# Autodesk Inventor assembly: Knee
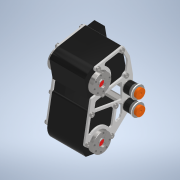
[picture p0: Inventor's stored thumbnail of the model, 180x180]
Saved by Autodesk Inventor 2020 (Build 240168000, 168)
## iProperties
Created: 2022-06-14
Part Number: Knee
Document SubType Name: Assembly
Designer: Masato Kubotera
Author: Masato Kubotera
## Documents named in this file (12)
- C:\Users\MasatoKubotera\Documents\Inventor\SUSTAINA-OP\LowerBody\Knee\Knee.iam
- C:\Users\MasatoKubotera\Documents\Inventor\SUSTAINA-OP\LowerBody\Knee\Knee_side_frame.ipt
- C:\Users\MasatoKubotera\Documents\Inventor\SUSTAINA-OP\ReadyMade\KONDO\B3M-SC-1170-A_with_ClampHorn_AND_FreeHorn.iam
- C:\Users\MasatoKubotera\Documents\Inventor\SUSTAINA-OP\ReadyMade\Screw\M2_6-15.ipt
- C:\Users\MasatoKubotera\Documents\Inventor\SUSTAINA-OP\ReadyMade\Spacer\SLSBF6-39.5-M4-N4.ipt
- C:\Users\MasatoKubotera\Documents\Inventor\SUSTAINA-OP\ReadyMade\Washer\UUW-0412-10H.ipt
- C:\Users\MasatoKubotera\Documents\Inventor\SUSTAINA-OP\ReadyMade\Washer\CCC-0612-65B.ipt
- C:\Users\MasatoKubotera\Documents\Inventor\SUSTAINA-OP\ReadyMade\Bush\80F-0603.ipt
- C:\Users\MasatoKubotera\Documents\Inventor\SUSTAINA-OP\ReadyMade\Screw\DBTS4-11-8-DHC.ipt
- C:\Users\MasatoKubotera\Documents\Inventor\SUSTAINA-OP\ReadyMade\Washer\UUW-0614-03H.ipt
- C:\Users\MasatoKubotera\Documents\Inventor\SUSTAINA-OP\ReadyMade\Washer\TT-0814-10.ipt
- C:\Users\MasatoKubotera\Documents\Inventor\SUSTAINA-OP\ReadyMade\Screw\M2_6-20.ipt
## Components (46 placed, 11 different names)
1. Knee_side_frame:1 — メイト:1, フラッシュ:2, 挿入:1, 挿入:2, 挿入:3, 挿入:4, 挿入:5, 挿入:6, 挿入:7, 挿入:8, 挿入:17, 挿入:18, 挿入:19, 挿入:20, 挿入:21, 挿入:22, 挿入:23, 挿入:24, 挿入:25, 挿入:26, 挿入:29, 挿入:30
2. Knee_side_frame:2 — 挿入:9, 挿入:10, 挿入:11, 挿入:12, 挿入:13, 挿入:14, 挿入:15, 挿入:16, 挿入:27, 挿入:28, 挿入:31, 挿入:32, 挿入:53, 挿入:54, 挿入:55, 挿入:56, 挿入:57, 挿入:58, 挿入:59, 挿入:60
3. B3M-SC-1170-A_with_ClampHorn_AND_FreeHorn:1 [sub-assembly] — フラッシュ:1, 挿入:1, 挿入:2, 挿入:3, 挿入:4, 挿入:9, 挿入:10, 挿入:11, 挿入:12
4. B3M-SC-1170-A_with_ClampHorn_AND_FreeHorn:2 [sub-assembly] — 挿入:5, 挿入:6, 挿入:7, 挿入:8, 挿入:13, 挿入:14, 挿入:15, 挿入:16
5. SLSBF6-39.5-M4-N4:1 — 挿入:25, 挿入:27
6. SLSBF6-39.5-M4-N4:2 — 挿入:26, 挿入:28
7. UUW-0412-10H:1 — 挿入:29, 挿入:33, 挿入:41
8. UUW-0412-10H:2 — 挿入:30, 挿入:34, 挿入:42
9. UUW-0412-10H:3 — 挿入:31, 挿入:35, 挿入:43
10. UUW-0412-10H:4 — 挿入:32, 挿入:36, 挿入:44
11. CCC-0612-65B:1 — 挿入:33, 挿入:37
12. CCC-0612-65B:2 — 挿入:34, 挿入:38
13. CCC-0612-65B:3 — 挿入:35, 挿入:39
14. CCC-0612-65B:4 — 挿入:36, 挿入:40
15. 80F-0603:1 — 挿入:37
16. 80F-0603:2 — 挿入:38
17. 80F-0603:3 — 挿入:39
18. 80F-0603:4 — 挿入:40
19. UUW-0614-03H:1 — 挿入:45, 挿入:50
20. UUW-0614-03H:2 — 挿入:46, 挿入:49
21. UUW-0614-03H:3 — 挿入:47, 挿入:51
22. UUW-0614-03H:4 — 挿入:48, 挿入:52
23. TT-0814-10:1 — 挿入:49
24. TT-0814-10:2 — 挿入:50
25. TT-0814-10:3 — 挿入:51
26. TT-0814-10:4 — 挿入:52
27. DBTS4-11-8-DHC:1 — 挿入:41, 挿入:46
28. DBTS4-11-8-DHC:2 — 挿入:42, 挿入:45
29. DBTS4-11-8-DHC:3 — 挿入:43, 挿入:47
30. DBTS4-11-8-DHC:4 — 挿入:44, 挿入:48
31. M2_6-15:1 — 挿入:17
32. M2_6-15:2 — 挿入:18
33. M2_6-15:3 — 挿入:20
34. M2_6-15:4 — 挿入:19
35. M2_6-15:5 — 挿入:21
36. M2_6-15:6 — 挿入:22
37. M2_6-15:7 — 挿入:23
38. M2_6-15:8 — 挿入:24
39. M2_6-20:1 — 挿入:53
40. M2_6-20:2 — 挿入:54
41. M2_6-20:3 — 挿入:55
42. M2_6-20:4 — 挿入:56
43. M2_6-20:5 — 挿入:57
44. M2_6-20:6 — 挿入:58
45. M2_6-20:7 — 挿入:59
46. M2_6-20:8 — 挿入:60
## Relationships (63: Insert 60, Flush 2, Mate 1)
- メイト:1 [Mate]: Knee_side_frame:1
- フラッシュ:1 [Flush] (21.75 mm): B3M-SC-1170-A_with_ClampHorn_AND_FreeHorn:1
- フラッシュ:2 [Flush]: Knee_side_frame:1
- 挿入:1 [Insert]: Knee_side_frame:1 ↔ B3M-SC-1170-A_with_ClampHorn_AND_FreeHorn:1
- 挿入:2 [Insert]: Knee_side_frame:1 ↔ B3M-SC-1170-A_with_ClampHorn_AND_FreeHorn:1
- 挿入:3 [Insert]: Knee_side_frame:1 ↔ B3M-SC-1170-A_with_ClampHorn_AND_FreeHorn:1
- 挿入:4 [Insert]: Knee_side_frame:1 ↔ B3M-SC-1170-A_with_ClampHorn_AND_FreeHorn:1
- 挿入:5 [Insert]: Knee_side_frame:1 ↔ B3M-SC-1170-A_with_ClampHorn_AND_FreeHorn:2
- 挿入:6 [Insert]: Knee_side_frame:1 ↔ B3M-SC-1170-A_with_ClampHorn_AND_FreeHorn:2
- 挿入:7 [Insert]: Knee_side_frame:1 ↔ B3M-SC-1170-A_with_ClampHorn_AND_FreeHorn:2
- 挿入:8 [Insert]: Knee_side_frame:1 ↔ B3M-SC-1170-A_with_ClampHorn_AND_FreeHorn:2
- 挿入:9 [Insert]: Knee_side_frame:2 ↔ B3M-SC-1170-A_with_ClampHorn_AND_FreeHorn:1
- 挿入:10 [Insert]: Knee_side_frame:2 ↔ B3M-SC-1170-A_with_ClampHorn_AND_FreeHorn:1
- 挿入:11 [Insert]: Knee_side_frame:2 ↔ B3M-SC-1170-A_with_ClampHorn_AND_FreeHorn:1
- 挿入:12 [Insert]: Knee_side_frame:2 ↔ B3M-SC-1170-A_with_ClampHorn_AND_FreeHorn:1
- 挿入:13 [Insert]: Knee_side_frame:2 ↔ B3M-SC-1170-A_with_ClampHorn_AND_FreeHorn:2
- 挿入:14 [Insert]: Knee_side_frame:2 ↔ B3M-SC-1170-A_with_ClampHorn_AND_FreeHorn:2
- 挿入:15 [Insert]: Knee_side_frame:2 ↔ B3M-SC-1170-A_with_ClampHorn_AND_FreeHorn:2
- 挿入:16 [Insert]: Knee_side_frame:2 ↔ B3M-SC-1170-A_with_ClampHorn_AND_FreeHorn:2
- 挿入:17 [Insert]: Knee_side_frame:1 ↔ M2_6-15:1
- 挿入:18 [Insert]: Knee_side_frame:1 ↔ M2_6-15:2
- 挿入:19 [Insert]: Knee_side_frame:1 ↔ M2_6-15:4
- 挿入:20 [Insert]: Knee_side_frame:1 ↔ M2_6-15:3
- 挿入:21 [Insert]: Knee_side_frame:1 ↔ M2_6-15:5
- 挿入:22 [Insert]: Knee_side_frame:1 ↔ M2_6-15:6
- 挿入:23 [Insert]: Knee_side_frame:1 ↔ M2_6-15:7
- 挿入:24 [Insert]: Knee_side_frame:1 ↔ M2_6-15:8
- 挿入:25 [Insert]: Knee_side_frame:1 ↔ SLSBF6-39.5-M4-N4:1
- 挿入:26 [Insert]: Knee_side_frame:1 ↔ SLSBF6-39.5-M4-N4:2
- 挿入:27 [Insert]: Knee_side_frame:2 ↔ SLSBF6-39.5-M4-N4:1
- 挿入:28 [Insert]: Knee_side_frame:2 ↔ SLSBF6-39.5-M4-N4:2
- 挿入:29 [Insert]: Knee_side_frame:1 ↔ UUW-0412-10H:1
- 挿入:30 [Insert]: Knee_side_frame:1 ↔ UUW-0412-10H:2
- 挿入:31 [Insert]: Knee_side_frame:2 ↔ UUW-0412-10H:3
- 挿入:32 [Insert]: Knee_side_frame:2 ↔ UUW-0412-10H:4
- 挿入:33 [Insert]: UUW-0412-10H:1 ↔ CCC-0612-65B:1
- 挿入:34 [Insert]: UUW-0412-10H:2 ↔ CCC-0612-65B:2
- 挿入:35 [Insert]: UUW-0412-10H:3 ↔ CCC-0612-65B:3
- 挿入:36 [Insert]: UUW-0412-10H:4 ↔ CCC-0612-65B:4
- 挿入:37 [Insert]: CCC-0612-65B:1 ↔ 80F-0603:1
- 挿入:38 [Insert]: CCC-0612-65B:2 ↔ 80F-0603:2
- 挿入:39 [Insert]: CCC-0612-65B:3 ↔ 80F-0603:3
- 挿入:40 [Insert]: CCC-0612-65B:4 ↔ 80F-0603:4
- 挿入:41 [Insert]: UUW-0412-10H:1 ↔ DBTS4-11-8-DHC:1
- 挿入:42 [Insert]: UUW-0412-10H:2 ↔ DBTS4-11-8-DHC:2
- 挿入:43 [Insert]: UUW-0412-10H:3 ↔ DBTS4-11-8-DHC:3
- 挿入:44 [Insert]: UUW-0412-10H:4 ↔ DBTS4-11-8-DHC:4
- 挿入:45 [Insert]: UUW-0614-03H:1 ↔ DBTS4-11-8-DHC:2
- 挿入:46 [Insert]: UUW-0614-03H:2 ↔ DBTS4-11-8-DHC:1
- 挿入:47 [Insert]: UUW-0614-03H:3 ↔ DBTS4-11-8-DHC:3
- 挿入:48 [Insert]: UUW-0614-03H:4 ↔ DBTS4-11-8-DHC:4
- 挿入:49 [Insert]: UUW-0614-03H:2 ↔ TT-0814-10:1
- 挿入:50 [Insert]: UUW-0614-03H:1 ↔ TT-0814-10:2
- 挿入:51 [Insert]: UUW-0614-03H:3 ↔ TT-0814-10:3
- 挿入:52 [Insert]: UUW-0614-03H:4 ↔ TT-0814-10:4
- 挿入:53 [Insert]: Knee_side_frame:2 ↔ M2_6-20:1
- 挿入:54 [Insert]: Knee_side_frame:2 ↔ M2_6-20:2
- 挿入:55 [Insert]: Knee_side_frame:2 ↔ M2_6-20:3
- 挿入:56 [Insert]: Knee_side_frame:2 ↔ M2_6-20:4
- 挿入:57 [Insert]: Knee_side_frame:2 ↔ M2_6-20:5
- 挿入:58 [Insert]: Knee_side_frame:2 ↔ M2_6-20:6
- 挿入:59 [Insert]: Knee_side_frame:2 ↔ M2_6-20:7
- 挿入:60 [Insert]: Knee_side_frame:2 ↔ M2_6-20:8
